# Autodesk Inventor assembly: 5v 18mm
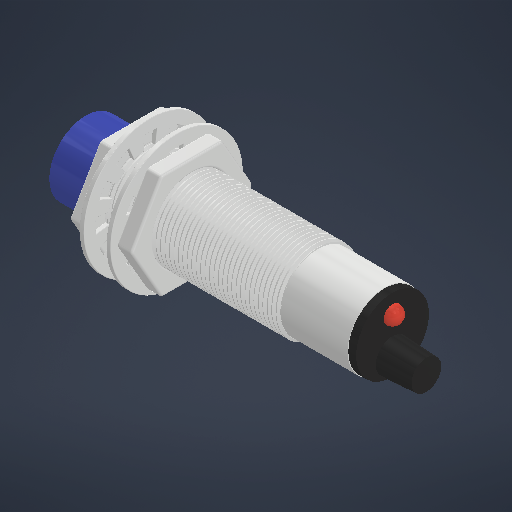
[picture p0: Inventor's stored thumbnail of the model, 512x512]
Saved by Autodesk Inventor 2027.1 (Build 311270010, 270A)
## iProperties
Created: 2020-10-23
Part Number: 5v 18mm
Document SubType Name: Assembly
Designer: daniel
Title: C:/Users/tempi/Documents/3D Printing/Inductive Proximity Sensor Assembly.step
Sending System: Autodesk Translation Framework v9.3.0.1241
Preprocessor: ST-DEVELOPER v18.1
## Documents named in this file (4)
- C:\Users\danda\Downloads\18mm-inductive-proximity-sensor-taiss-bed-leveling-sensor-1.snapshot.4\Inductive Proximity Sensor Assembly\Inductive Proximity Sensor Assembly.iam
- C:\Users\danda\Downloads\18mm-inductive-proximity-sensor-taiss-bed-leveling-sensor-1.snapshot.4\Inductive Proximity Sensor Assembly\Sensor.ipt
- C:\Users\danda\Downloads\18mm-inductive-proximity-sensor-taiss-bed-leveling-sensor-1.snapshot.4\Inductive Proximity Sensor Assembly\Nut.ipt
- C:\Users\danda\Downloads\18mm-inductive-proximity-sensor-taiss-bed-leveling-sensor-1.snapshot.4\Inductive Proximity Sensor Assembly\Lock Washer.ipt
## Components (5 placed, 3 different names)
1. Sensor:1 — Mate:7, Flush:1
2. Nut:1 — Mate:2, Mate:4, Mate:6, Flush:1
3. Nut:2 — Mate:3, Mate:4, Mate:7
4. Lock Washer:1 — Mate:1, Mate:2, Mate:5, Mate:6
5. Lock Washer:2 — Mate:1, Mate:3, Mate:5
## Relationships (8: Mate 7, Flush 1)
- Mate:1 (5 mm): Lock Washer:1 ↔ Lock Washer:2
- Mate:2: Nut:1 ↔ Lock Washer:1
- Mate:3: Nut:2 ↔ Lock Washer:2
- Mate:4: Nut:1 ↔ Nut:2
- Mate:5: Lock Washer:1 ↔ Lock Washer:2
- Mate:6: Nut:1 ↔ Lock Washer:1
- Mate:7: Sensor:1 ↔ Nut:2
- Flush:1 (10 mm): Sensor:1 ↔ Nut:1
